# Autodesk Inventor assembly: Content Center
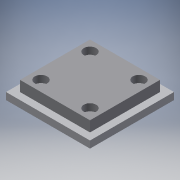
[picture p0: Inventor's stored thumbnail of the model, 180x180]
Saved by Autodesk Inventor 2016 (Build 200138000, 138)
## iProperties
Created: 2014-03-06
Part Number: Content Center
Document SubType Name: Assembly
Designer: John
Author: John
## Documents named in this file (3)
- C:\File Storage\Autodesk\Inventor 2016 Projects\Ex_Files_Inventor_2016_EssT\Exercise Files\14_Adding parts to an assembly file\14_04\Content Center.iam
- C:\File Storage\Autodesk\Inventor 2016 Projects\Ex_Files_Inventor_2016_EssT\Exercise Files\14_Adding parts to an assembly file\14_04\Base Plate.ipt
- C:\File Storage\Autodesk\Inventor 2016 Projects\Ex_Files_Inventor_2016_EssT\Exercise Files\14_Adding parts to an assembly file\14_04\Block.ipt
## Components (2 placed, 2 different names)
1. Base Plate:1 — Mate:1, Mate:2, Mate:3
2. Block:1 — Mate:1, Mate:2, Mate:3
## Relationships (3: Mate 3)
- Mate:1: Base Plate:1 ↔ Block:1
- Mate:2: Base Plate:1 ↔ Block:1
- Mate:3: Base Plate:1 ↔ Block:1
